# Autodesk Inventor assembly: motor
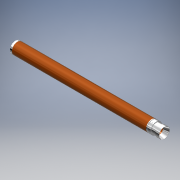
[picture p0: Inventor's stored thumbnail of the model, 180x180]
Saved by Autodesk Inventor 2017 SP1 (Build 210196100, 196)
## iProperties
Created: 2016-10-29
Part Number: motor
Document SubType Name: Assembly
Designer: cflannery
Author: cflannery
## Documents named in this file (6)
- D:\Triton_Rocket_Club\Propulsion\Launches\8-inch-flight\Design\CAD\Vehicle\Structures\motor.iam
- D:\Triton_Rocket_Club\Propulsion\Launches\8-inch-flight\Design\CAD\Vehicle\Structures\phenolic_liner.ipt
- D:\Triton_Rocket_Club\Propulsion\Launches\8-inch-flight\Design\CAD\Vehicle\Structures\thermal_barrier.ipt
- D:\Triton_Rocket_Club\Propulsion\Launches\8-inch-flight\Design\CAD\Vehicle\Nozzle\trunk\nozzle.iam
- D:\Triton_Rocket_Club\Propulsion\Launches\8-inch-flight\Design\CAD\Vehicle\Structures\filled_casting_tube.iam
- D:\Triton_Rocket_Club\Propulsion\Launches\8-inch-flight\Design\CAD\Vehicle\Structures\motor_bulkhead.ipt
## Components (10 placed, 5 different names)
1. phenolic_liner:1 — Mate:34, Mate:38, Mate:40, Mate:42
2. filled_casting_tube:1 [sub-assembly] — Mate:23, Mate:24, Mate:25, Mate:29, Mate:30
3. filled_casting_tube:2 [sub-assembly] — Mate:23, Mate:28, Mate:29
4. filled_casting_tube:3 [sub-assembly] — Mate:24, Mate:28, Mate:41
5. filled_casting_tube:4 [sub-assembly] — Mate:25, Mate:26, Mate:31, Mate:32
6. filled_casting_tube:5 [sub-assembly] — Mate:26, Mate:27, Mate:30, Mate:31, Mate:34
7. filled_casting_tube:6 [sub-assembly] — Mate:27, Mate:32, Mate:36, Mate:37
8. thermal_barrier:1 — Mate:37, Mate:38, Mate:39
9. motor_bulkhead:1 — Mate:36, Mate:39
10. nozzle:1 [sub-assembly] — Mate:40, Mate:41, Mate:42
## Relationships (18: Mate 18)
- Mate:23: filled_casting_tube:1 ↔ filled_casting_tube:2
- Mate:24: filled_casting_tube:1 ↔ filled_casting_tube:3
- Mate:25: filled_casting_tube:1 ↔ filled_casting_tube:4
- Mate:26: filled_casting_tube:4 ↔ filled_casting_tube:5
- Mate:27: filled_casting_tube:5 ↔ filled_casting_tube:6
- Mate:28: filled_casting_tube:2 ↔ filled_casting_tube:3
- Mate:29: filled_casting_tube:1 ↔ filled_casting_tube:2
- Mate:30: filled_casting_tube:1 ↔ filled_casting_tube:5
- Mate:31: filled_casting_tube:4 ↔ filled_casting_tube:5
- Mate:32: filled_casting_tube:4 ↔ filled_casting_tube:6
- Mate:34: phenolic_liner:1 ↔ filled_casting_tube:5
- Mate:36: filled_casting_tube:6 ↔ motor_bulkhead:1
- Mate:37: filled_casting_tube:6 ↔ thermal_barrier:1
- Mate:38: phenolic_liner:1 ↔ thermal_barrier:1
- Mate:39: thermal_barrier:1 ↔ motor_bulkhead:1
- Mate:40: phenolic_liner:1 ↔ nozzle:1
- Mate:41: filled_casting_tube:3 ↔ nozzle:1
- Mate:42: phenolic_liner:1 ↔ nozzle:1
